# Autodesk Inventor assembly: motormounttempassem
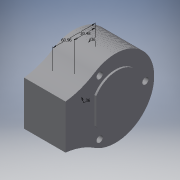
[picture p0: Inventor's stored thumbnail of the model, 180x180]
Saved by Autodesk Inventor 2019 (Build 230136000, 136)
## iProperties
Created: 2018-08-02
Part Number: motormounttempassem
Document SubType Name: Assembly
Designer: Kitte_X
Author: Kitte_X
## Documents named in this file (3)
- C:\Users\Kitte_X\Documents\Inventor\BattleBot\motormounttempassem.iam
- C:\Users\Kitte_X\Documents\Inventor\BattleBot\battlebotmotorbracetemp.ipt
- C:\Users\Kitte_X\Documents\Inventor\BattleBot\BattleBotmotormock.ipt
## Components (21 placed, 2 different names)
1. BattleBotmotormock:1 — Mate:1, Mate:2, Flush:1
2. battlebotmotorbracetemp:1 — Mate:1, Mate:2, Flush:1
3. battlebotmotorbracetemp:2
4. battlebotmotorbracetemp:3
5. battlebotmotorbracetemp:4
6. battlebotmotorbracetemp:5
7. battlebotmotorbracetemp:6
8. battlebotmotorbracetemp:7
9. battlebotmotorbracetemp:8
10. battlebotmotorbracetemp:9
11. battlebotmotorbracetemp:10
12. battlebotmotorbracetemp:11
13. battlebotmotorbracetemp:12
14. battlebotmotorbracetemp:13
15. battlebotmotorbracetemp:14
16. battlebotmotorbracetemp:15
17. battlebotmotorbracetemp:16
18. battlebotmotorbracetemp:17
19. battlebotmotorbracetemp:18
20. battlebotmotorbracetemp:19
21. battlebotmotorbracetemp:20
## Component patterns: (20 elements, first: battlebotmotorbracetemp:1)
## Relationships (3: Mate 2, Flush 1)
- Mate:1: BattleBotmotormock:1 ↔ battlebotmotorbracetemp:1
- Mate:2: BattleBotmotormock:1 ↔ battlebotmotorbracetemp:1
- Flush:1: BattleBotmotormock:1 ↔ battlebotmotorbracetemp:1
